# Autodesk Inventor assembly: Сборка
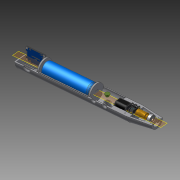
[picture p0: Inventor's stored thumbnail of the model, 180x180]
Saved by Autodesk Inventor 2014 (Build 180170000, 170)
## iProperties
Created: 2017-11-09
Part Number: Сборка
Document SubType Name: Assembly
Designer: Nikopol
Author: Nikopol
## Documents named in this file (10)
- D:\Inventor\otvertka\Сборка.iam
- D:\Inventor\otvertka\korpus_1.ipt
- D:\Inventor\otvertka\TP4056.ipt
- D:\Inventor\otvertka\gear motorIGS.ipt
- D:\Inventor\otvertka\623zz\roulement_623-2z_0.iam
- D:\Inventor\otvertka\Battery 18650.ipt
- D:\Inventor\otvertka\Vtulka.ipt
- D:\Inventor\otvertka\korpus_2.ipt
- D:\Inventor\otvertka\pwr_btn.ipt
- D:\Inventor\otvertka\btn.ipt
## Components (9 placed, 9 different names)
1. korpus_1:1 — Совмещение:1, Совмещение:2, Совмещение:3, Совмещение:4, Совмещение:5, Совмещение:7, Совмещение:8, Совмещение:9, Заподлицо:1, Вставка:1
2. TP4056:1 — Совмещение:1, Совмещение:2
3. gear motorIGS:1 — Совмещение:7, Совмещение:8
4. roulement_623-2z_0:1 [sub-assembly] — Совмещение:4, Совмещение:5, Касательность:1, Совмещение:6
5. Battery 18650:1 — Совмещение:3
6. Vtulka:1 — Касательность:1, Совмещение:6
7. korpus_2:1 — Совмещение:9, Заподлицо:1
8. pwr_btn:1
9. btn:1 — Вставка:1
## Relationships (12: Mate 9, Tangent 1, Flush 1, Insert 1)
- Совмещение:1 [Mate]: korpus_1:1 ↔ TP4056:1
- Совмещение:2 [Mate]: korpus_1:1 ↔ TP4056:1
- Совмещение:3 [Mate]: korpus_1:1 ↔ Battery 18650:1
- Совмещение:4 [Mate]: korpus_1:1 ↔ roulement_623-2z_0:1
- Совмещение:5 [Mate]: korpus_1:1 ↔ roulement_623-2z_0:1
- Касательность:1 [Tangent]: roulement_623-2z_0:1 ↔ Vtulka:1
- Совмещение:6 [Mate] (0.1 mm): roulement_623-2z_0:1 ↔ Vtulka:1
- Совмещение:7 [Mate]: korpus_1:1 ↔ gear motorIGS:1
- Совмещение:8 [Mate]: korpus_1:1 ↔ gear motorIGS:1
- Совмещение:9 [Mate]: korpus_1:1 ↔ korpus_2:1
- Заподлицо:1 [Flush]: korpus_1:1 ↔ korpus_2:1
- Вставка:1 [Insert] (10 mm): korpus_1:1 ↔ btn:1
